# Autodesk Inventor assembly: Rocker-Bogie-Robot-ASM-01
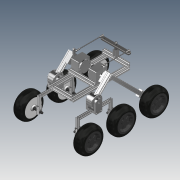
[picture p0: Inventor's stored thumbnail of the model, 180x180]
Saved by Autodesk Inventor 2018.2 (Build 222227000, 227)
## iProperties
Manager: feesmrt
Company: FRANCOR
Created: 2017-12-16
Part Number: Rocker-Bogie-Robot-ASM-01
Material: Generisch
Document SubType Name: Assembly
Designer: feesmrt
Project: Rescue Robot
Cost Center: -
Description: Rocker Bogie Robot Ver 01
Engineer: feesmrt
Authority: feesmrt
Stock Number: Rocker-Bogie-Robot-ASM-01
Author: feesmrt
Title: Rocker Bogie Robot Ver 01
Subject: Rescue Robot
Revision Number: 1
## Documents named in this file (11)
- D:\Programmierung\FRANC0R\CAD\02-Rocker-Bogie-Robot\Rocker-Bogie-Robot-ASM-01.iam
- D:\Programmierung\FRANC0R\CAD\02-Rocker-Bogie-Robot\100-CHASSIS\100-CHASSIS-ASM-01.iam
- D:\Programmierung\FRANC0R\CAD\02-Rocker-Bogie-Robot\200-ROCKER-BOGIE\200-10-ROCKER-BEARING\200-10-ROCKER-BEARING-ASM-01.iam
- D:\Programmierung\FRANC0R\CAD\02-Rocker-Bogie-Robot\200-ROCKER-BOGIE\200-02-ROCKER-CONNECTOR-ASM-L.iam
- D:\Programmierung\FRANC0R\CAD\02-Rocker-Bogie-Robot\200-ROCKER-BOGIE\200-02-ROCKER-CONNECTOR-ASM-R.iam
- D:\Programmierung\FRANC0R\CAD\02-Rocker-Bogie-Robot\200-ROCKER-BOGIE\200-03-BOGIE-CONNECTOR-ASM.iam
- D:\Programmierung\FRANC0R\CAD\02-Rocker-Bogie-Robot\900-COMPONENTS\900-10-WHEEL\900-10-WHEEL-ASM-01.iam
- D:\Programmierung\FRANC0R\CAD\02-Rocker-Bogie-Robot\200-ROCKER-BOGIE\200-60-DIFFERENTIAL\200-60-DIFFERENTIAL-CONNECTOR-01.iam
- D:\Programmierung\FRANC0R\CAD\02-Rocker-Bogie-Robot\200-ROCKER-BOGIE\200-60-DIFFERENTIAL\200-60-DIFFERENTIAL-CONNECTOR-02.iam
- D:\Programmierung\FRANC0R\CAD\02-Rocker-Bogie-Robot\200-ROCKER-BOGIE\200-60-DIFFERENTIAL\200-60-DIFFERENTIAL-BAR-L-01.iam
- D:\Programmierung\FRANC0R\CAD\02-Rocker-Bogie-Robot\200-ROCKER-BOGIE\200-60-DIFFERENTIAL\200-60-DIFFERENTIAL-BAR-R-01.iam
## Components (17 placed, 10 different names)
1. 100-CHASSIS-ASM-01:1 [sub-assembly] — Passend:27, Passend:29, Passend:30, Passend:31, Fluchtend:1, Passend:32
2. 200-10-ROCKER-BEARING-ASM-01:1 [sub-assembly] — Passend:7, Passend:8, Passend:29, Passend:30
3. 200-10-ROCKER-BEARING-ASM-01:2 [sub-assembly] — Passend:9, Passend:10, Passend:27, Passend:31
4. 200-02-ROCKER-CONNECTOR-ASM-L:1 [sub-assembly] — Passend:7, Passend:8, Passend:11, Passend:12, Passend:19, Winkel:7, Passend:20, Passend:36
5. 200-02-ROCKER-CONNECTOR-ASM-R:1 [sub-assembly] — Passend:9, Passend:10, Winkel:2, Passend:13, Passend:14, Passend:21, Winkel:8, Passend:22, Passend:38
6. 200-03-BOGIE-CONNECTOR-ASM:1 [sub-assembly] — Passend:11, Passend:12, Winkel:3, Passend:15, Winkel:5, Passend:16, Passend:17, Passend:18, Winkel:6
7. 200-03-BOGIE-CONNECTOR-ASM:2 [sub-assembly] — Passend:13, Passend:14, Winkel:4, Passend:23, Winkel:9, Passend:24, Passend:25, Passend:26, Winkel:10
8. 900-10-WHEEL-ASM-01:1 [sub-assembly] — Passend:15, Winkel:5, Passend:16
9. 900-10-WHEEL-ASM-01:2 [sub-assembly] — Passend:17, Passend:18, Winkel:6
10. 900-10-WHEEL-ASM-01:3 [sub-assembly] — Passend:19, Winkel:7, Passend:20
11. 900-10-WHEEL-ASM-01:4 [sub-assembly] — Passend:21, Winkel:8, Passend:22
12. 900-10-WHEEL-ASM-01:5 [sub-assembly] — Passend:23, Winkel:9, Passend:24
13. 900-10-WHEEL-ASM-01:6 [sub-assembly] — Passend:25, Passend:26, Winkel:10
14. 200-60-DIFFERENTIAL-CONNECTOR-01:1 [sub-assembly] — Fluchtend:1, Passend:32, Fluchtend:2, Passend:33, Passend:34
15. 200-60-DIFFERENTIAL-CONNECTOR-02:1 [sub-assembly] — Passend:33, Passend:34, Passend:35, Passend:37
16. 200-60-DIFFERENTIAL-BAR-L-01:1 [sub-assembly] — Passend:35, Passend:36
17. 200-60-DIFFERENTIAL-BAR-R-01:1 [sub-assembly] — Passend:37, Passend:38
## Relationships (42: Mate 31, Angle 9, Flush 2)
- Passend:7 [Mate]: 200-10-ROCKER-BEARING-ASM-01:1 ↔ 200-02-ROCKER-CONNECTOR-ASM-L:1
- Passend:8 [Mate]: 200-10-ROCKER-BEARING-ASM-01:1 ↔ 200-02-ROCKER-CONNECTOR-ASM-L:1
- Passend:9 [Mate]: 200-10-ROCKER-BEARING-ASM-01:2 ↔ 200-02-ROCKER-CONNECTOR-ASM-R:1
- Passend:10 [Mate]: 200-10-ROCKER-BEARING-ASM-01:2 ↔ 200-02-ROCKER-CONNECTOR-ASM-R:1
- Winkel:2 [Angle] (0 deg): 200-02-ROCKER-CONNECTOR-ASM-R:1
- Passend:11 [Mate]: 200-02-ROCKER-CONNECTOR-ASM-L:1 ↔ 200-03-BOGIE-CONNECTOR-ASM:1
- Passend:12 [Mate]: 200-02-ROCKER-CONNECTOR-ASM-L:1 ↔ 200-03-BOGIE-CONNECTOR-ASM:1
- Passend:13 [Mate]: 200-02-ROCKER-CONNECTOR-ASM-R:1 ↔ 200-03-BOGIE-CONNECTOR-ASM:2
- Passend:14 [Mate]: 200-02-ROCKER-CONNECTOR-ASM-R:1 ↔ 200-03-BOGIE-CONNECTOR-ASM:2
- Winkel:3 [Angle] (0 deg): 200-03-BOGIE-CONNECTOR-ASM:1
- Winkel:4 [Angle] (0 deg): 200-03-BOGIE-CONNECTOR-ASM:2
- Passend:15 [Mate]: 200-03-BOGIE-CONNECTOR-ASM:1 ↔ 900-10-WHEEL-ASM-01:1
- Winkel:5 [Angle] (0 deg): 200-03-BOGIE-CONNECTOR-ASM:1 ↔ 900-10-WHEEL-ASM-01:1
- Passend:16 [Mate] (5 mm): 200-03-BOGIE-CONNECTOR-ASM:1 ↔ 900-10-WHEEL-ASM-01:1
- Passend:17 [Mate]: 200-03-BOGIE-CONNECTOR-ASM:1 ↔ 900-10-WHEEL-ASM-01:2
- Passend:18 [Mate] (5 mm): 200-03-BOGIE-CONNECTOR-ASM:1 ↔ 900-10-WHEEL-ASM-01:2
- Winkel:6 [Angle] (0 deg): 200-03-BOGIE-CONNECTOR-ASM:1 ↔ 900-10-WHEEL-ASM-01:2
- Passend:19 [Mate]: 200-02-ROCKER-CONNECTOR-ASM-L:1 ↔ 900-10-WHEEL-ASM-01:3
- Winkel:7 [Angle] (0 deg): 200-02-ROCKER-CONNECTOR-ASM-L:1 ↔ 900-10-WHEEL-ASM-01:3
- Passend:20 [Mate]: 200-02-ROCKER-CONNECTOR-ASM-L:1 ↔ 900-10-WHEEL-ASM-01:3
- Passend:21 [Mate]: 200-02-ROCKER-CONNECTOR-ASM-R:1 ↔ 900-10-WHEEL-ASM-01:4
- Winkel:8 [Angle] (0 deg): 200-02-ROCKER-CONNECTOR-ASM-R:1 ↔ 900-10-WHEEL-ASM-01:4
- Passend:22 [Mate]: 200-02-ROCKER-CONNECTOR-ASM-R:1 ↔ 900-10-WHEEL-ASM-01:4
- Passend:23 [Mate]: 200-03-BOGIE-CONNECTOR-ASM:2 ↔ 900-10-WHEEL-ASM-01:5
- Winkel:9 [Angle] (0 deg): 200-03-BOGIE-CONNECTOR-ASM:2 ↔ 900-10-WHEEL-ASM-01:5
- Passend:24 [Mate] (5 mm): 200-03-BOGIE-CONNECTOR-ASM:2 ↔ 900-10-WHEEL-ASM-01:5
- Passend:25 [Mate]: 200-03-BOGIE-CONNECTOR-ASM:2 ↔ 900-10-WHEEL-ASM-01:6
- Passend:26 [Mate] (5 mm): 200-03-BOGIE-CONNECTOR-ASM:2 ↔ 900-10-WHEEL-ASM-01:6
- Winkel:10 [Angle] (0 deg): 200-03-BOGIE-CONNECTOR-ASM:2 ↔ 900-10-WHEEL-ASM-01:6
- Passend:27 [Mate]: 100-CHASSIS-ASM-01:1 ↔ 200-10-ROCKER-BEARING-ASM-01:2
- Passend:29 [Mate]: 100-CHASSIS-ASM-01:1 ↔ 200-10-ROCKER-BEARING-ASM-01:1
- Passend:30 [Mate]: 100-CHASSIS-ASM-01:1 ↔ 200-10-ROCKER-BEARING-ASM-01:1
- Passend:31 [Mate]: 100-CHASSIS-ASM-01:1 ↔ 200-10-ROCKER-BEARING-ASM-01:2
- Fluchtend:1 [Flush]: 100-CHASSIS-ASM-01:1 ↔ 200-60-DIFFERENTIAL-CONNECTOR-01:1
- Passend:32 [Mate]: 100-CHASSIS-ASM-01:1 ↔ 200-60-DIFFERENTIAL-CONNECTOR-01:1
- Fluchtend:2 [Flush]: 200-60-DIFFERENTIAL-CONNECTOR-01:1
- Passend:33 [Mate]: 200-60-DIFFERENTIAL-CONNECTOR-01:1 ↔ 200-60-DIFFERENTIAL-CONNECTOR-02:1
- Passend:34 [Mate]: 200-60-DIFFERENTIAL-CONNECTOR-01:1 ↔ 200-60-DIFFERENTIAL-CONNECTOR-02:1
- Passend:35 [Mate]: 200-60-DIFFERENTIAL-CONNECTOR-02:1 ↔ 200-60-DIFFERENTIAL-BAR-L-01:1
- Passend:36 [Mate]: 200-02-ROCKER-CONNECTOR-ASM-L:1 ↔ 200-60-DIFFERENTIAL-BAR-L-01:1
- Passend:37 [Mate]: 200-60-DIFFERENTIAL-CONNECTOR-02:1 ↔ 200-60-DIFFERENTIAL-BAR-R-01:1
- Passend:38 [Mate]: 200-02-ROCKER-CONNECTOR-ASM-R:1 ↔ 200-60-DIFFERENTIAL-BAR-R-01:1
## Named parameters: Angle_Rocker = 0 deg, Angle_Bogie_Left = 0 deg, Angle_Bogie_Right = 0 deg
